# Autodesk Inventor assembly: CLB_048_FourPartScissorHalf
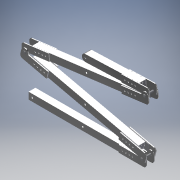
[picture p0: Inventor's stored thumbnail of the model, 180x180]
Saved by Autodesk Inventor 2018.3 (Build 223284000, 284)
## iProperties
Created: 2020-02-13
Part Number: CLB_048_FourPartScissorHalf
Document SubType Name: Assembly
Designer: Cooper
Author: Cooper
## Documents named in this file (9)
- C:\Users\22perngrac\Documents\GrabCAD\Infinite Recharge 2020\Build season\CLB_048_FourPartScissorHalf.iam
- C:\Users\22perngrac\Documents\GrabCAD\Infinite Recharge 2020\Build season\CLB_036_FourPartScissorBarTop.ipt
- C:\Users\22perngrac\Documents\GrabCAD\Infinite Recharge 2020\Build season\CLB_027_LifterBracket.ipt
- C:\Users\22perngrac\Documents\GrabCAD\Infinite Recharge 2020\Build season\CLB_040_ScissorLiftSpacer2.ipt
- C:\Users\22perngrac\Documents\GrabCAD\Infinite Recharge 2020\Build season\CLB_046_ClevisPinScissors.ipt
- C:\Users\22perngrac\Documents\GrabCAD\Infinite Recharge 2020\Build season\CLB_053_ScissorTopBarPlug.ipt
- C:\Users\22perngrac\Documents\GrabCAD\Infinite Recharge 2020\Build season\CLB_052_ScissorLiftPlug.ipt
- C:\Users\22perngrac\Documents\GrabCAD\Infinite Recharge 2020\Build season\CLB_042_BottomBarFourPartScissors.ipt
- C:\Users\22perngrac\Documents\GrabCAD\Infinite Recharge 2020\Build season\CLB_049_MiddleBarFourPartScissors.ipt
## Components (32 placed, 8 different names)
1. CLB_042_BottomBarFourPartScissors:1 — Mate:3, Flush:2, Mate:4, Flush:3, Flush:4, Mate:25, Angle:1, Mate:45, Mate:46, Flush:50, Flush:51
2. CLB_049_MiddleBarFourPartScissors:1 — Mate:5, Mate:6, Flush:8, Flush:9, Flush:12, Flush:14, Flush:16, Mate:10, Mate:11, Flush:17, Flush:18, Flush:19, Flush:20, Flush:22, Flush:23, Mate:25, Mate:26, Mate:41, Mate:42, Flush:48, Mate:43, Mate:44, Flush:49, Flush:51
3. CLB_049_MiddleBarFourPartScissors:2 — Flush:16, Mate:14, Flush:24, Flush:25, Mate:15, Flush:26, Flush:27, Mate:17, Mate:18, Flush:28, Flush:29, Flush:30, Flush:31, Flush:33, Flush:34, Mate:26, Mate:27, Flush:43, Mate:36, Mate:37, Flush:46, Mate:38, Mate:39, Mate:40, Flush:47
4. CLB_036_FourPartScissorBarTop:1 — Mate:21, Mate:22, Flush:37, Flush:38, Flush:39, Flush:40, Mate:27, Flush:43, Mate:31, Mate:32, Flush:44, Mate:33, Flush:45, Mate:34, Mate:35
5. CLB_027_LifterBracket:1 — Mate:3, Flush:2, Mate:29, Angle:1
6. CLB_027_LifterBracket:2 — Mate:8, Flush:12, Flush:13, Insert:3
7. CLB_027_LifterBracket:3 — Mate:7, Flush:10, Flush:14, Flush:15, Mate:30
8. CLB_027_LifterBracket:4 — Mate:4, Flush:3, Flush:4, Mate:28
9. CLB_027_LifterBracket:5 — Mate:12, Flush:19, Flush:20, Flush:21
10. CLB_027_LifterBracket:6 — Mate:15, Flush:26, Flush:27
11. CLB_027_LifterBracket:7 — Mate:14, Flush:24, Flush:25, Mate:16
12. CLB_027_LifterBracket:8 — Mate:13, Flush:22, Flush:23, Mate:16, Flush:41, Insert:2
13. CLB_027_LifterBracket:9 — Mate:22, Flush:38, Flush:40, Mate:23
14. CLB_027_LifterBracket:10 — Mate:21, Flush:37, Flush:39
15. CLB_027_LifterBracket:11 — Mate:20, Flush:33, Flush:34, Flush:35, Insert:1
16. CLB_027_LifterBracket:12 — Mate:19, Flush:30, Flush:31, Flush:32, Mate:23
17. CLB_040_ScissorLiftSpacer2:1 — Mate:6, Flush:8, Mate:8, Flush:13
18. CLB_040_ScissorLiftSpacer2:2 — Mate:5, Flush:9, Mate:7, Flush:15, Flush:10
19. CLB_040_ScissorLiftSpacer2:3 — Mate:11, Flush:18, Mate:13, Flush:41
20. CLB_040_ScissorLiftSpacer2:4 — Mate:10, Flush:17, Mate:12, Flush:21
21. CLB_040_ScissorLiftSpacer2:5 — Mate:18, Flush:29, Mate:20, Flush:35
22. CLB_040_ScissorLiftSpacer2:6 — Mate:17, Flush:28, Mate:19, Flush:32
23. CLB_046_ClevisPinScissors:1 — Insert:3, Mate:28, Mate:29, Mate:30
24. CLB_046_ClevisPinScissors:2 — Insert:2
25. CLB_046_ClevisPinScissors:3 — Insert:1
26. CLB_053_ScissorTopBarPlug:1 — Mate:31, Mate:32, Flush:44
27. CLB_052_ScissorLiftPlug:1 — Mate:36, Mate:37, Flush:46, Mate:38
28. CLB_052_ScissorLiftPlug:2 — Mate:33, Flush:45, Mate:34, Mate:35
29. CLB_052_ScissorLiftPlug:3 — Mate:39, Mate:40, Flush:47
30. CLB_052_ScissorLiftPlug:4 — Mate:41, Mate:42, Flush:48
31. CLB_052_ScissorLiftPlug:5 — Mate:43, Mate:44, Flush:49
32. CLB_052_ScissorLiftPlug:6 — Mate:45, Mate:46, Flush:50
## Relationships (90: Flush 44, Mate 42, Insert 3, Angle 1)
- Mate:3: CLB_042_BottomBarFourPartScissors:1 ↔ CLB_027_LifterBracket:1
- Flush:2 (-38.1 mm): CLB_042_BottomBarFourPartScissors:1 ↔ CLB_027_LifterBracket:1
- Mate:4: CLB_042_BottomBarFourPartScissors:1 ↔ CLB_027_LifterBracket:4
- Flush:3: CLB_042_BottomBarFourPartScissors:1 ↔ CLB_027_LifterBracket:4
- Flush:4 (-38.1 mm): CLB_042_BottomBarFourPartScissors:1 ↔ CLB_027_LifterBracket:4
- Mate:5: CLB_049_MiddleBarFourPartScissors:1 ↔ CLB_040_ScissorLiftSpacer2:2
- Mate:6: CLB_049_MiddleBarFourPartScissors:1 ↔ CLB_040_ScissorLiftSpacer2:1
- Flush:8: CLB_049_MiddleBarFourPartScissors:1 ↔ CLB_040_ScissorLiftSpacer2:1
- Flush:9: CLB_049_MiddleBarFourPartScissors:1 ↔ CLB_040_ScissorLiftSpacer2:2
- Mate:7: CLB_027_LifterBracket:3 ↔ CLB_040_ScissorLiftSpacer2:2
- Flush:10: CLB_027_LifterBracket:3 ↔ CLB_040_ScissorLiftSpacer2:2
- Mate:8: CLB_027_LifterBracket:2 ↔ CLB_040_ScissorLiftSpacer2:1
- Flush:12 (-38.1 mm): CLB_049_MiddleBarFourPartScissors:1 ↔ CLB_027_LifterBracket:2
- Flush:13: CLB_027_LifterBracket:2 ↔ CLB_040_ScissorLiftSpacer2:1
- Flush:14 (-38.1 mm): CLB_049_MiddleBarFourPartScissors:1 ↔ CLB_027_LifterBracket:3
- Flush:15: CLB_027_LifterBracket:3 ↔ CLB_040_ScissorLiftSpacer2:2
- Flush:16: CLB_049_MiddleBarFourPartScissors:1 ↔ CLB_049_MiddleBarFourPartScissors:2
- Mate:10: CLB_049_MiddleBarFourPartScissors:1 ↔ CLB_040_ScissorLiftSpacer2:4
- Mate:11: CLB_049_MiddleBarFourPartScissors:1 ↔ CLB_040_ScissorLiftSpacer2:3
- Flush:17: CLB_049_MiddleBarFourPartScissors:1 ↔ CLB_040_ScissorLiftSpacer2:4
- Flush:18: CLB_049_MiddleBarFourPartScissors:1 ↔ CLB_040_ScissorLiftSpacer2:3
- Mate:12: CLB_027_LifterBracket:5 ↔ CLB_040_ScissorLiftSpacer2:4
- Flush:19: CLB_049_MiddleBarFourPartScissors:1 ↔ CLB_027_LifterBracket:5
- Flush:20 (-38.1 mm): CLB_049_MiddleBarFourPartScissors:1 ↔ CLB_027_LifterBracket:5
- Flush:21: CLB_027_LifterBracket:5 ↔ CLB_040_ScissorLiftSpacer2:4
- Mate:13: CLB_027_LifterBracket:8 ↔ CLB_040_ScissorLiftSpacer2:3
- Flush:22: CLB_049_MiddleBarFourPartScissors:1 ↔ CLB_027_LifterBracket:8
- Flush:23 (-38.1 mm): CLB_049_MiddleBarFourPartScissors:1 ↔ CLB_027_LifterBracket:8
- Mate:14: CLB_049_MiddleBarFourPartScissors:2 ↔ CLB_027_LifterBracket:7
- Flush:24: CLB_049_MiddleBarFourPartScissors:2 ↔ CLB_027_LifterBracket:7
- Flush:25 (-38.1 mm): CLB_049_MiddleBarFourPartScissors:2 ↔ CLB_027_LifterBracket:7
- Mate:15: CLB_049_MiddleBarFourPartScissors:2 ↔ CLB_027_LifterBracket:6
- Flush:26: CLB_049_MiddleBarFourPartScissors:2 ↔ CLB_027_LifterBracket:6
- Flush:27 (-38.1 mm): CLB_049_MiddleBarFourPartScissors:2 ↔ CLB_027_LifterBracket:6
- Mate:16: CLB_027_LifterBracket:7 ↔ CLB_027_LifterBracket:8
- Mate:17: CLB_049_MiddleBarFourPartScissors:2 ↔ CLB_040_ScissorLiftSpacer2:6
- Mate:18: CLB_049_MiddleBarFourPartScissors:2 ↔ CLB_040_ScissorLiftSpacer2:5
- Flush:28: CLB_049_MiddleBarFourPartScissors:2 ↔ CLB_040_ScissorLiftSpacer2:6
- Flush:29: CLB_049_MiddleBarFourPartScissors:2 ↔ CLB_040_ScissorLiftSpacer2:5
- Mate:19: CLB_027_LifterBracket:12 ↔ CLB_040_ScissorLiftSpacer2:6
- Flush:30: CLB_049_MiddleBarFourPartScissors:2 ↔ CLB_027_LifterBracket:12
- Flush:31 (-38.1 mm): CLB_049_MiddleBarFourPartScissors:2 ↔ CLB_027_LifterBracket:12
- Flush:32: CLB_027_LifterBracket:12 ↔ CLB_040_ScissorLiftSpacer2:6
- Mate:20: CLB_027_LifterBracket:11 ↔ CLB_040_ScissorLiftSpacer2:5
- Flush:33: CLB_049_MiddleBarFourPartScissors:2 ↔ CLB_027_LifterBracket:11
- Flush:34 (-38.1 mm): CLB_049_MiddleBarFourPartScissors:2 ↔ CLB_027_LifterBracket:11
- Flush:35: CLB_027_LifterBracket:11 ↔ CLB_040_ScissorLiftSpacer2:5
- Mate:21: CLB_036_FourPartScissorBarTop:1 ↔ CLB_027_LifterBracket:10
- Mate:22: CLB_036_FourPartScissorBarTop:1 ↔ CLB_027_LifterBracket:9
- Flush:37: CLB_036_FourPartScissorBarTop:1 ↔ CLB_027_LifterBracket:10
- Flush:38: CLB_036_FourPartScissorBarTop:1 ↔ CLB_027_LifterBracket:9
- Flush:39 (-38.1 mm): CLB_036_FourPartScissorBarTop:1 ↔ CLB_027_LifterBracket:10
- Flush:40 (-38.1 mm): CLB_036_FourPartScissorBarTop:1 ↔ CLB_027_LifterBracket:9
- Mate:23: CLB_027_LifterBracket:9 ↔ CLB_027_LifterBracket:12
- Insert:1: CLB_027_LifterBracket:11 ↔ CLB_046_ClevisPinScissors:3
- Insert:2: CLB_027_LifterBracket:8 ↔ CLB_046_ClevisPinScissors:2
- Insert:3: CLB_027_LifterBracket:2 ↔ CLB_046_ClevisPinScissors:1
- Flush:41: CLB_027_LifterBracket:8 ↔ CLB_040_ScissorLiftSpacer2:3
- Mate:25: CLB_042_BottomBarFourPartScissors:1 ↔ CLB_049_MiddleBarFourPartScissors:1
- Mate:26: CLB_049_MiddleBarFourPartScissors:1 ↔ CLB_049_MiddleBarFourPartScissors:2
- Mate:27: CLB_049_MiddleBarFourPartScissors:2 ↔ CLB_036_FourPartScissorBarTop:1
- Flush:43: CLB_049_MiddleBarFourPartScissors:2 ↔ CLB_036_FourPartScissorBarTop:1
- Mate:28: CLB_027_LifterBracket:4 ↔ CLB_046_ClevisPinScissors:1
- Mate:29: CLB_027_LifterBracket:1 ↔ CLB_046_ClevisPinScissors:1
- Mate:30: CLB_027_LifterBracket:3 ↔ CLB_046_ClevisPinScissors:1
- Angle:1 (0 deg): CLB_042_BottomBarFourPartScissors:1 ↔ CLB_027_LifterBracket:1
- Mate:31: CLB_036_FourPartScissorBarTop:1 ↔ CLB_053_ScissorTopBarPlug:1
- Mate:32: CLB_036_FourPartScissorBarTop:1 ↔ CLB_053_ScissorTopBarPlug:1
- Flush:44 (176.2125 mm): CLB_036_FourPartScissorBarTop:1 ↔ CLB_053_ScissorTopBarPlug:1
- Mate:33: CLB_036_FourPartScissorBarTop:1 ↔ CLB_052_ScissorLiftPlug:2
- Flush:45: CLB_036_FourPartScissorBarTop:1 ↔ CLB_052_ScissorLiftPlug:2
- Mate:34: CLB_036_FourPartScissorBarTop:1 ↔ CLB_052_ScissorLiftPlug:2
- Mate:35: CLB_036_FourPartScissorBarTop:1 ↔ CLB_052_ScissorLiftPlug:2
- Mate:36: CLB_049_MiddleBarFourPartScissors:2 ↔ CLB_052_ScissorLiftPlug:1
- Mate:37: CLB_049_MiddleBarFourPartScissors:2 ↔ CLB_052_ScissorLiftPlug:1
- Flush:46: CLB_049_MiddleBarFourPartScissors:2 ↔ CLB_052_ScissorLiftPlug:1
- Mate:38: CLB_049_MiddleBarFourPartScissors:2 ↔ CLB_052_ScissorLiftPlug:1
- Mate:39: CLB_049_MiddleBarFourPartScissors:2 ↔ CLB_052_ScissorLiftPlug:3
- Mate:40: CLB_049_MiddleBarFourPartScissors:2 ↔ CLB_052_ScissorLiftPlug:3
- Flush:47: CLB_049_MiddleBarFourPartScissors:2 ↔ CLB_052_ScissorLiftPlug:3
- Mate:41: CLB_049_MiddleBarFourPartScissors:1 ↔ CLB_052_ScissorLiftPlug:4
- Mate:42: CLB_049_MiddleBarFourPartScissors:1 ↔ CLB_052_ScissorLiftPlug:4
- Flush:48: CLB_049_MiddleBarFourPartScissors:1 ↔ CLB_052_ScissorLiftPlug:4
- Mate:43: CLB_049_MiddleBarFourPartScissors:1 ↔ CLB_052_ScissorLiftPlug:5
- Mate:44: CLB_049_MiddleBarFourPartScissors:1 ↔ CLB_052_ScissorLiftPlug:5
- Flush:49: CLB_049_MiddleBarFourPartScissors:1 ↔ CLB_052_ScissorLiftPlug:5
- Mate:45: CLB_042_BottomBarFourPartScissors:1 ↔ CLB_052_ScissorLiftPlug:6
- Mate:46: CLB_042_BottomBarFourPartScissors:1 ↔ CLB_052_ScissorLiftPlug:6
- Flush:50: CLB_042_BottomBarFourPartScissors:1 ↔ CLB_052_ScissorLiftPlug:6
- Flush:51: CLB_042_BottomBarFourPartScissors:1 ↔ CLB_049_MiddleBarFourPartScissors:1
